# Autodesk Inventor assembly: Plstic Box Rear A Assembly with Battery Spacers
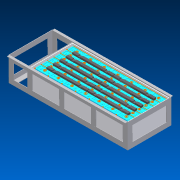
[picture p0: Inventor's stored thumbnail of the model, 180x180]
Saved by Autodesk Inventor 2012 (Build 160160000, 160)
## iProperties
Created: 2012-07-02
Part Number: Plstic Box Rear A Assembly with Battery Spacers
Document SubType Name: Assembly
Designer: Hemant
Author: Hemant
## Documents named in this file (4)
- C:\Users\Hemant\Documents\Pastic Box - Rear A\Plstic Box Rear A Assembly with Battery Spacers.iam
- C:\Users\Hemant\Documents\Battery Box C Assembly.iam
- C:\Users\Hemant\Documents\Pastic Box - Rear A\Batteries Pack New.iam
- C:\Users\Hemant\Documents\Pastic Box - Rear A\spacer 1.ipt
## Components (12 placed, 3 different names)
1. Battery Box C Assembly:1 [sub-assembly] — Mate:16, Mate:17, Mate:18
2. Batteries Pack New:1 [sub-assembly] — Mate:16, Mate:17, Mate:18, Mate:19, Mate:20
3. spacer 1:1 — Mate:19
4. spacer 1:2
5. spacer 1:3
6. spacer 1:4
7. spacer 1:5
8. spacer 1:6
9. spacer 1:7
10. spacer 1:8
11. spacer 1:9 — Mate:20
12. spacer 1:10
## Component patterns: (10 elements, first: spacer 1:1)
## Relationships (5: Mate 5)
- Mate:16: Battery Box C Assembly:1 ↔ Batteries Pack New:1
- Mate:17: Battery Box C Assembly:1 ↔ Batteries Pack New:1
- Mate:18: Battery Box C Assembly:1 ↔ Batteries Pack New:1
- Mate:19: Batteries Pack New:1 ↔ spacer 1:1
- Mate:20 (73.66 mm): Batteries Pack New:1 ↔ spacer 1:9
